# Autodesk Inventor assembly: DriveChain V3
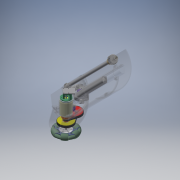
[picture p0: Inventor's stored thumbnail of the model, 180x180]
Saved by Autodesk Inventor 2019.1 (Build 231200000, 200)
## iProperties
Created: 2018-11-14
Part Number: DriveChain V3
Material: Generisch
Document SubType Name: Assembly
Designer: JochenAlt
Author: JochenAlt
## Documents named in this file (11)
- D:\Projects\Ondine\CAD\DriveChain V3.iam
- D:\Projects\Ondine\CAD\DriveChainEnclosure V3.ipt
- D:\Projects\Ondine\CAD\Beltdrive\BeltGear.iam
- D:\Projects\Ondine\CAD\Bearings\W 637_4 X-2Z.iam
- D:\Projects\Ondine\CAD\OmniWheel.iam
- D:\Projects\Ondine\CAD\BushOmniWheelV3.ipt
- D:\Projects\Ondine\CAD\BeltDriveAxisV3.ipt
- D:\Projects\Ondine\CAD\Leg\Worm.iam
- D:\Projects\Ondine\CAD\Leg\LegRod.iam
- D:\Projects\Ondine\CAD\Bearings\W 617_3.iam
- D:\Projects\Ondine\CAD\Leg\Leg V4.iam
## Components (15 placed, 10 different names)
1. DriveChainEnclosure:1 — Passend:1, Passend:2, Passend:3, Passend:12, Passend:14, Passend:15, Passend:16, Passend:17, Passend:42, Passend:43, Passend:44, Passend:45, Passend:46, Passend:47, Passend:54, Passend:55
2. NewBeltGear:1 [sub-assembly] — Passend:20, Passend:21, Passend:26
3. W 637_4 X-2Z:1 [sub-assembly] — Passend:1, Passend:2, Passend:20, Passend:21
4. W 637_4 X-2Z:2 [sub-assembly] — Passend:3, Passend:16, Passend:23
5. OmniWheel:1 [sub-assembly] — Passend:18, Passend:19
6. BushOmniWheel:1 — Passend:12, Passend:17, Passend:18, Passend:19
7. W 637_4 X-2Z:3 [sub-assembly] — Passend:14, Passend:15, Passend:22
8. HarmonicDrive-Axis:1 — Passend:22, Passend:23, Passend:26
9. Worm:1 [sub-assembly] — Passend:42, Passend:43, Passend:48, Passend:49, Passend:50, Drehung:1
10. LegRod:1 [sub-assembly] — Passend:44, Passend:45, Passend:51, Passend:52, Passend:53, Drehung:1
11. W 617_3:1 [sub-assembly] — Passend:46, Passend:51
12. W 617_3:2 [sub-assembly] — Passend:47, Passend:50
13. W 617_3:3 [sub-assembly] — Passend:48, Passend:49
14. W 617_3:4 [sub-assembly] — Passend:52, Passend:53
15. Leg V4:1 [sub-assembly] — Passend:54, Passend:55
## Relationships (30: Mate 29, RelateRotation 1)
- Passend:1 [Mate]: DriveChainEnclosure:1 ↔ W 637_4 X-2Z:1
- Passend:2 [Mate]: DriveChainEnclosure:1 ↔ W 637_4 X-2Z:1
- Passend:3 [Mate]: DriveChainEnclosure:1 ↔ W 637_4 X-2Z:2
- Passend:12 [Mate]: DriveChainEnclosure:1 ↔ BushOmniWheel:1
- Passend:14 [Mate]: DriveChainEnclosure:1 ↔ W 637_4 X-2Z:3
- Passend:15 [Mate]: DriveChainEnclosure:1 ↔ W 637_4 X-2Z:3
- Passend:16 [Mate]: DriveChainEnclosure:1 ↔ W 637_4 X-2Z:2
- Passend:17 [Mate]: DriveChainEnclosure:1 ↔ BushOmniWheel:1
- Passend:18 [Mate]: OmniWheel:1 ↔ BushOmniWheel:1
- Passend:19 [Mate]: OmniWheel:1 ↔ BushOmniWheel:1
- Passend:20 [Mate]: NewBeltGear:1 ↔ W 637_4 X-2Z:1
- Passend:21 [Mate]: NewBeltGear:1 ↔ W 637_4 X-2Z:1
- Passend:22 [Mate]: W 637_4 X-2Z:3 ↔ HarmonicDrive-Axis:1
- Passend:23 [Mate]: W 637_4 X-2Z:2 ↔ HarmonicDrive-Axis:1
- Passend:26 [Mate]: NewBeltGear:1 ↔ HarmonicDrive-Axis:1
- Passend:42 [Mate]: DriveChainEnclosure:1 ↔ Worm:1
- Passend:43 [Mate]: DriveChainEnclosure:1 ↔ Worm:1
- Passend:44 [Mate]: DriveChainEnclosure:1 ↔ LegRod:1
- Passend:45 [Mate]: DriveChainEnclosure:1 ↔ LegRod:1
- Passend:46 [Mate]: DriveChainEnclosure:1 ↔ W 617_3:1
- Passend:47 [Mate]: DriveChainEnclosure:1 ↔ W 617_3:2
- Passend:48 [Mate]: Worm:1 ↔ W 617_3:3
- Passend:49 [Mate]: Worm:1 ↔ W 617_3:3
- Passend:50 [Mate]: Worm:1 ↔ W 617_3:2
- Passend:51 [Mate]: LegRod:1 ↔ W 617_3:1
- Passend:52 [Mate]: LegRod:1 ↔ W 617_3:4
- Passend:53 [Mate]: LegRod:1 ↔ W 617_3:4
- Drehung:1 [RelateRotation] (1 ul): Worm:1 ↔ LegRod:1
- Passend:54 [Mate]: DriveChainEnclosure:1 ↔ Leg V4:1
- Passend:55 [Mate]: DriveChainEnclosure:1 ↔ Leg V4:1
